# Autodesk Inventor assembly: Paddleboat
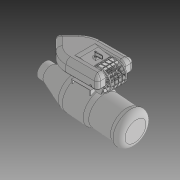
[picture p0: Inventor's stored thumbnail of the model, 180x180]
Saved by Autodesk Inventor 2020 (Build 240168000, 168)
## iProperties
Created: 2021-05-05
Part Number: Paddleboat
Document SubType Name: Assembly
Designer: DDeGo
Author: DDeGo
## Documents named in this file (17)
- C:\Users\DDeGo\Documents\Drew\Projects\AirWankelEngine\cad\Paddleboat\Paddleboat.iam
- C:\Users\DDeGo\Documents\Drew\Projects\AirWankelEngine\cad\Paddleboat\Hull.ipt
- C:\Users\DDeGo\Documents\Drew\Projects\AirWankelEngine\cad\Paddleboat\688 bearing.ipt
- C:\Users\DDeGo\Documents\Drew\Projects\AirWankelEngine\cad\Paddleboat\Paddlewheel.ipt
- C:\Users\DDeGo\Documents\Drew\Projects\AirWankelEngine\cad\Paddleboat\Rudder.ipt
- C:\Users\DDeGo\Documents\Drew\Projects\AirWankelEngine\cad\Paddleboat\PaddleRotatingZone.ipt
- C:\Users\DDeGo\Documents\Drew\Projects\AirWankelEngine\cad\IntegzaVersion\Wankel_Engine_Assy.iam
- C:\Users\DDeGo\Documents\Drew\Projects\AirWankelEngine\cad\Paddleboat\ServoArm.ipt
- C:\Users\DDeGo\Documents\Drew\Projects\AirWankelEngine\cad\Paddleboat\MG90servo_body.ipt
- C:\Users\DDeGo\Documents\Drew\Projects\AirWankelEngine\cad\Paddleboat\Deck.ipt
- C:\Users\DDeGo\Documents\Drew\Projects\AirWankelEngine\cad\Paddleboat\2L bottle.ipt
- C:\Users\DDeGo\Documents\Drew\Projects\AirWankelEngine\cad\Paddleboat\DrivenPulley.ipt
- C:\Users\DDeGo\Documents\Drew\Projects\AirWankelEngine\cad\Paddleboat\DrivePulley.ipt
- C:\Users\DDeGo\Documents\Drew\Projects\AirWankelEngine\cad\Paddleboat\Rubberband.ipt
- C:\Users\DDeGo\Documents\Drew\Projects\AirWankelEngine\cad\Paddleboat\ServoHorn.ipt
- C:\Users\DDeGo\Documents\Drew\Projects\AirWankelEngine\cad\Paddleboat\ServoLink.ipt
- C:\Users\DDeGo\Documents\Drew\Projects\AirWankelEngine\cad\MiniRegulator\Regulator.iam
## Components (17 placed, 16 different names)
1. Hull:1 — Mate:1, Mate:2, Flush:1, Flush:2, Mate:6, Mate:7, Mate:10, Mate:11, Mate:13, Mate:14, Mate:15, Mate:17, Mate:18, Mate:19, Mate:20, Mate:21, Mate:22, Flush:4, Mate:23
2. 688 bearing:1 — Mate:2, Flush:2, Mate:8
3. Paddlewheel:1 — Mate:8, Mate:9, Mate:12, Flush:3, Flush:5
4. Rudder:1 — Mate:6, Mate:7, Angle:1, Angle:2
5. 688 bearing:2 — Mate:1, Flush:1, Mate:9, Mate:25, Mate:26
6. PaddleRotatingZone:1 — Mate:12, Flush:3
7. Wankel_Engine_Assy:1 [sub-assembly] — Mate:13, Mate:14, Mate:15, Mate:27, Mate:28, Mate:29
8. ServoArm:1 — Mate:17, Angle:2, Mate:21, Mate:35
9. MG90servo_body:1 — Mate:18, Mate:19, Mate:20, Mate:32, Mate:33
10. Deck:1 — Mate:22, Flush:4, Mate:23, Mate:37, Mate:38
11. 2L bottle:1 — Mate:37, Mate:38
12. DrivenPulley:1 — Mate:25, Mate:26, Rotation:1, Flush:5, Mate:36
13. DrivePulley:1 — Mate:27, Rotation:1, Mate:28, Mate:29
14. Rubberband:1 — Mate:36
15. ServoHorn:1 — Mate:32, Mate:33, Mate:34
16. ServoLink:1 — Mate:34, Mate:35
17. Regulator:1 [sub-assembly]
## Relationships (39: Mate 31, Flush 5, Angle 2, RelateRotation 1)
- Mate:1: Hull:1 ↔ 688 bearing:2
- Mate:2: Hull:1 ↔ 688 bearing:1
- Flush:1: Hull:1 ↔ 688 bearing:2
- Flush:2: Hull:1 ↔ 688 bearing:1
- Mate:6: Hull:1 ↔ Rudder:1
- Mate:7: Hull:1 ↔ Rudder:1
- Mate:8: 688 bearing:1 ↔ Paddlewheel:1
- Mate:9 (1.5 mm): Paddlewheel:1 ↔ 688 bearing:2
- Angle:1 (180 deg): Rudder:1
- Mate:10: Hull:1
- Mate:11: Hull:1
- Mate:12: Paddlewheel:1 ↔ PaddleRotatingZone:1
- Flush:3 (-1 mm): Paddlewheel:1 ↔ PaddleRotatingZone:1
- Mate:13: Hull:1 ↔ Wankel_Engine_Assy:1
- Mate:14: Hull:1 ↔ Wankel_Engine_Assy:1
- Mate:15: Hull:1 ↔ Wankel_Engine_Assy:1
- Mate:17: Hull:1 ↔ ServoArm:1
- Angle:2 (-60 deg): Rudder:1 ↔ ServoArm:1
- Mate:18: Hull:1 ↔ MG90servo_body:1
- Mate:19: Hull:1 ↔ MG90servo_body:1
- Mate:20: Hull:1 ↔ MG90servo_body:1
- Mate:21: Hull:1 ↔ ServoArm:1
- Mate:22: Hull:1 ↔ Deck:1
- Flush:4: Hull:1 ↔ Deck:1
- Mate:23: Hull:1 ↔ Deck:1
- Mate:25: 688 bearing:2 ↔ DrivenPulley:1
- Mate:26: 688 bearing:2 ↔ DrivenPulley:1
- Mate:27: Wankel_Engine_Assy:1 ↔ DrivePulley:1
- Rotation:1 [RelateRotation] (5.143 ul): DrivenPulley:1 ↔ DrivePulley:1
- Mate:28 (1.5 mm): Wankel_Engine_Assy:1 ↔ DrivePulley:1
- Flush:5: Paddlewheel:1 ↔ DrivenPulley:1
- Mate:29: Wankel_Engine_Assy:1 ↔ DrivePulley:1
- Mate:32: MG90servo_body:1 ↔ ServoHorn:1
- Mate:33: MG90servo_body:1 ↔ ServoHorn:1
- Mate:34: ServoHorn:1 ↔ ServoLink:1
- Mate:35: ServoArm:1 ↔ ServoLink:1
- Mate:36: DrivenPulley:1 ↔ Rubberband:1
- Mate:37: Deck:1 ↔ 2L bottle:1
- Mate:38: Deck:1 ↔ 2L bottle:1
